# Autodesk Inventor assembly: Gameboy NG
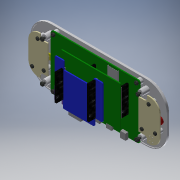
[picture p0: Inventor's stored thumbnail of the model, 180x180]
Saved by Autodesk Inventor 2019 (Build 230136000, 136)
## iProperties
Created: 2018-06-05
Part Number: Gameboy NG
Material: Générique
Document SubType Name: Assembly
Designer: dimercur
Author: dimercur
## Documents named in this file (13)
- D:\Users\dimercur\Documents locaux\Travail\git\arm-ada-ng\hardware\Box\Gameboy NG.iam
- D:\Users\dimercur\Documents locaux\Travail\git\arm-ada-ng\hardware\Box\STM32F746G-Disco.ipt
- D:\Users\dimercur\Documents locaux\Travail\git\arm-ada-ng\hardware\Box\Partie Haute.ipt
- D:\Users\dimercur\Documents locaux\Travail\git\arm-ada-ng\hardware\Box\Button.ipt
- D:\Users\dimercur\Documents locaux\Travail\git\arm-ada-ng\hardware\Box\Cross.ipt
- D:\Users\dimercur\Documents locaux\Travail\git\arm-ada-ng\hardware\Box\Partie basse.ipt
- D:\Users\dimercur\Documents locaux\Travail\git\arm-ada-ng\hardware\Box\Satellite Gauche.iam
- D:\Users\dimercur\Documents locaux\Travail\git\arm-ada-ng\hardware\Box\Satellite Droit.iam
- D:\Users\dimercur\Documents locaux\Travail\git\arm-ada-ng\hardware\Box\X-Nucleo-IKS01A1.ipt
- D:\Users\dimercur\Documents locaux\Travail\git\arm-ada-ng\hardware\Box\PCB Wifi.ipt
- U:\Inventor\Content Center Files\R2019\fr-FR\ISO 7045  H\ISO 7045 - M3 x 8 - 4.8 - H - ISO.ipt
- U:\Inventor\Content Center Files\R2019\fr-FR\ISO 7045  Z\ISO 7045 - M2,5 x 3 - 4.8 - Z - ISO.ipt
- U:\Inventor\Content Center Files\R2019\fr-FR\ISO 7045  Z\ISO 7045 - M3 x 4 - 4.8 - Z - ISO.ipt
## Components (26 placed, 12 different names)
1. STM32F746G-Disco:1 — Placage:1, Placage:2, Placage:3, Placage:27, Placage:28, Placage:29, Logement:11, Logement:12, Logement:13, Logement:14
2. Partie Haute:1 — Placage:1, Placage:2, Placage:3, Affleurement:1, Placage:4, Placage:6, Placage:8, Placage:9, Placage:10, Placage:11, Placage:12, Placage:13, Placage:14, Placage:15, Placage:16, Placage:17, Placage:18, Placage:19, Placage:20, Placage:21, Placage:22, Placage:23, Placage:24, Placage:25, Placage:26
3. Button:1 — Placage:9, Placage:14
4. Button:2 — Placage:6, Placage:10
5. Button:3 — Placage:11, Placage:13
6. Button:4 — Placage:8, Placage:12
7. Cross:1 — Placage:15, Placage:16, Placage:17
8. Dessous:1 — Placage:18, Placage:19, Placage:20, Logement:1, Logement:2, Logement:3, Logement:4
9. Satellite Gauche:1 [sub-assembly] — Placage:21, Placage:22, Placage:23, Logement:5, Logement:6, Logement:7
10. Satellite Droit:1 [sub-assembly] — Placage:24, Placage:25, Placage:26, Logement:8, Logement:9, Logement:10
11. X-Nucleo-IKS01A1:1 — Placage:30, Placage:31, Placage:32
12. PCB Wifi:1 — Placage:27, Placage:28, Placage:29, Placage:30, Placage:31, Placage:32
13. ISO 7045 H M3 x 8 - 4.8 - H:1 — Logement:1
14. ISO 7045 H M3 x 8 - 4.8 - H:2 — Logement:2
15. ISO 7045 H M3 x 8 - 4.8 - H:3 — Logement:3
16. ISO 7045 H M3 x 8 - 4.8 - H:4 — Logement:4
17. ISO 7045 Z M2,5 x 3 - 4.8 - Z:1 — Logement:5
18. ISO 7045 Z M2,5 x 3 - 4.8 - Z:2 — Logement:6
19. ISO 7045 Z M2,5 x 3 - 4.8 - Z:3 — Logement:7
20. ISO 7045 Z M2,5 x 3 - 4.8 - Z:4 — Logement:8
21. ISO 7045 Z M2,5 x 3 - 4.8 - Z:5 — Logement:9
22. ISO 7045 Z M2,5 x 3 - 4.8 - Z:6 — Logement:10
23. ISO 7045 Z M3 x 4 - 4.8 - Z:1 — Logement:11
24. ISO 7045 Z M3 x 4 - 4.8 - Z:2 — Logement:12
25. ISO 7045 Z M3 x 4 - 4.8 - Z:3 — Logement:13
26. ISO 7045 Z M3 x 4 - 4.8 - Z:4 — Logement:14
## Relationships (45: Mate 30, Insert 14, Flush 1)
- Placage:1 [Mate]: STM32F746G-Disco:1 ↔ Partie Haute:1
- Placage:2 [Mate]: STM32F746G-Disco:1 ↔ Partie Haute:1
- Placage:3 [Mate]: STM32F746G-Disco:1 ↔ Partie Haute:1
- Affleurement:1 [Flush]: Partie Haute:1
- Placage:4 [Mate]: Partie Haute:1
- Placage:6 [Mate]: Partie Haute:1 ↔ Button:2
- Placage:8 [Mate]: Partie Haute:1 ↔ Button:4
- Placage:9 [Mate]: Partie Haute:1 ↔ Button:1
- Placage:10 [Mate]: Partie Haute:1 ↔ Button:2
- Placage:11 [Mate]: Partie Haute:1 ↔ Button:3
- Placage:12 [Mate]: Partie Haute:1 ↔ Button:4
- Placage:13 [Mate]: Partie Haute:1 ↔ Button:3
- Placage:14 [Mate]: Partie Haute:1 ↔ Button:1
- Placage:15 [Mate]: Partie Haute:1 ↔ Cross:1
- Placage:16 [Mate] (0.5 mm): Partie Haute:1 ↔ Cross:1
- Placage:17 [Mate] (0.5 mm): Partie Haute:1 ↔ Cross:1
- Placage:18 [Mate]: Partie Haute:1 ↔ Dessous:1
- Placage:19 [Mate]: Partie Haute:1 ↔ Dessous:1
- Placage:20 [Mate]: Partie Haute:1 ↔ Dessous:1
- Placage:21 [Mate]: Partie Haute:1 ↔ Satellite Gauche:1
- Placage:22 [Mate]: Partie Haute:1 ↔ Satellite Gauche:1
- Placage:23 [Mate]: Partie Haute:1 ↔ Satellite Gauche:1
- Placage:24 [Mate]: Partie Haute:1 ↔ Satellite Droit:1
- Placage:25 [Mate]: Partie Haute:1 ↔ Satellite Droit:1
- Placage:26 [Mate]: Partie Haute:1 ↔ Satellite Droit:1
- Placage:27 [Mate]: STM32F746G-Disco:1 ↔ PCB Wifi:1
- Placage:28 [Mate]: STM32F746G-Disco:1 ↔ PCB Wifi:1
- Placage:29 [Mate]: STM32F746G-Disco:1 ↔ PCB Wifi:1
- Placage:30 [Mate]: X-Nucleo-IKS01A1:1 ↔ PCB Wifi:1
- Placage:31 [Mate]: X-Nucleo-IKS01A1:1 ↔ PCB Wifi:1
- Placage:32 [Mate]: X-Nucleo-IKS01A1:1 ↔ PCB Wifi:1
- Logement:1 [Insert]: Dessous:1 ↔ ISO 7045 H M3 x 8 - 4.8 - H:1
- Logement:2 [Insert]: Dessous:1 ↔ ISO 7045 H M3 x 8 - 4.8 - H:2
- Logement:3 [Insert]: Dessous:1 ↔ ISO 7045 H M3 x 8 - 4.8 - H:3
- Logement:4 [Insert]: Dessous:1 ↔ ISO 7045 H M3 x 8 - 4.8 - H:4
- Logement:5 [Insert]: Satellite Gauche:1 ↔ ISO 7045 Z M2,5 x 3 - 4.8 - Z:1
- Logement:6 [Insert]: Satellite Gauche:1 ↔ ISO 7045 Z M2,5 x 3 - 4.8 - Z:2
- Logement:7 [Insert]: Satellite Gauche:1 ↔ ISO 7045 Z M2,5 x 3 - 4.8 - Z:3
- Logement:8 [Insert]: Satellite Droit:1 ↔ ISO 7045 Z M2,5 x 3 - 4.8 - Z:4
- Logement:9 [Insert]: Satellite Droit:1 ↔ ISO 7045 Z M2,5 x 3 - 4.8 - Z:5
- Logement:10 [Insert]: Satellite Droit:1 ↔ ISO 7045 Z M2,5 x 3 - 4.8 - Z:6
- Logement:11 [Insert]: STM32F746G-Disco:1 ↔ ISO 7045 Z M3 x 4 - 4.8 - Z:1
- Logement:12 [Insert]: STM32F746G-Disco:1 ↔ ISO 7045 Z M3 x 4 - 4.8 - Z:2
- Logement:13 [Insert]: STM32F746G-Disco:1 ↔ ISO 7045 Z M3 x 4 - 4.8 - Z:3
- Logement:14 [Insert]: STM32F746G-Disco:1 ↔ ISO 7045 Z M3 x 4 - 4.8 - Z:4
